# Autodesk Inventor assembly: Frame
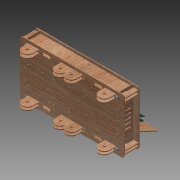
[picture p0: Inventor's stored thumbnail of the model, 180x180]
Saved by Autodesk Inventor 2015 (Build 190159000, 159)
## iProperties
Created: 2015-12-19
Part Number: Frame
Document SubType Name: Assembly
Designer: david
Author: david
## Documents named in this file (8)
- Z:\gip\Inventor\generatie 7\Frame\Frame.iam
- Z:\gip\Inventor\generatie 7\Frame\Electronica\Electronica.iam
- Z:\gip\Inventor\generatie 7\Frame\doos\zijiplaaten.ipt
- Z:\gip\Inventor\generatie 7\Frame\doos\voor-plaat.ipt
- Z:\gip\Inventor\generatie 7\Frame\afscherming.iam
- Z:\gip\Inventor\generatie 7\Frame\doos\TussenPalet.ipt
- Z:\gip\Inventor\generatie 7\Frame\vijs\vijs.ipt
- Z:\gip\Inventor\generatie 7\Frame\vijs\Moer.ipt
## Components (17 placed, 7 different names)
1. zijiplaaten:1 — Mate:26, Mate:35, Angle:1
2. zijiplaaten:2 — Mate:27
3. zijiplaaten:3 — Mate:20, Mate:36, Flush:3
4. zijiplaaten:4 — Mate:29, Mate:30, Mate:31, Flush:2
5. voor-plaat:1 — Flush:1, Mate:33
6. voor-plaat:2 — Mate:30, Mate:31, Mate:34
7. Electronica:1 [sub-assembly] — Mate:26, Mate:27, Mate:29, Mate:37, Mate:50, Mate:52, Mate:54, Mate:56
8. afscherming:1 [sub-assembly] — Mate:20, Mate:35, Mate:36, Flush:2, Flush:3, Mate:38, Mate:39, Mate:41, Mate:43, Mate:44, Mate:45, Mate:48
9. TussenPalet:1 — Flush:1, Mate:33, Mate:34
10. vijs:1 — Mate:37, Mate:38, Mate:49
11. vijs:2 — Mate:39, Mate:41, Mate:55
12. vijs:4 — Mate:43, Mate:44, Mate:51
13. vijs:5 — Mate:45, Mate:48, Mate:53
14. Moer:1 — Mate:49, Mate:50, Angle:1
15. Moer:2 — Mate:51, Mate:52
16. Moer:3 — Mate:53, Mate:54
17. Moer:4 — Mate:55, Mate:56
## Relationships (42: Mate 38, Flush 3, Angle 1)
- [Mate]: zijiplaaten:1 ↔ Electronica:1
- [Mate]: zijiplaaten:1 ↔ Electronica:1
- [Mate] (0.25 mm): zijiplaaten:2 ↔ Electronica:1
- [Mate] (2 mm): zijiplaaten:2 ↔ Electronica:1
- [Mate]: zijiplaaten:2 ↔ Electronica:1
- [Mate]: zijiplaaten:3 ↔ Electronica:1
- [Mate]: zijiplaaten:4 ↔ Electronica:1
- [Mate]: zijiplaaten:4 ↔ Electronica:1
- [Mate] (0.25 mm): zijiplaaten:1 ↔ voor-plaat:1
- [Mate] (0.25 mm): zijiplaaten:1 ↔ voor-plaat:1
- [Mate]: voor-plaat:1 ↔ Electronica:1
- [Mate]: voor-plaat:2 ↔ Electronica:1
- Mate:20: zijiplaaten:3 ↔ afscherming:1
- Mate:26 (2 mm): zijiplaaten:1 ↔ Electronica:1
- Mate:27 (2 mm): zijiplaaten:2 ↔ Electronica:1
- Mate:29 (2 mm): zijiplaaten:4 ↔ Electronica:1
- Mate:30 (0.25 mm): zijiplaaten:4 ↔ voor-plaat:2
- Mate:31 (0.25 mm): zijiplaaten:4 ↔ voor-plaat:2
- Flush:1: voor-plaat:1 ↔ TussenPalet:1
- Mate:33 (1 mm): voor-plaat:1 ↔ TussenPalet:1
- Mate:34: voor-plaat:2 ↔ TussenPalet:1
- Mate:35 (0.15 mm): zijiplaaten:1 ↔ afscherming:1
- Mate:36 (0.15 mm): zijiplaaten:3 ↔ afscherming:1
- Flush:2: zijiplaaten:4 ↔ afscherming:1
- Flush:3: zijiplaaten:3 ↔ afscherming:1
- Mate:37: Electronica:1 ↔ vijs:1
- Mate:38: afscherming:1 ↔ vijs:1
- Mate:39: afscherming:1 ↔ vijs:2
- Mate:41: afscherming:1 ↔ vijs:2
- Mate:43: afscherming:1 ↔ vijs:4
- Mate:44: afscherming:1 ↔ vijs:4
- Mate:45: afscherming:1 ↔ vijs:5
- Mate:48: afscherming:1 ↔ vijs:5
- Mate:49: vijs:1 ↔ Moer:1
- Mate:50: Electronica:1 ↔ Moer:1
- Angle:1 (0 deg): zijiplaaten:1 ↔ Moer:1
- Mate:51: vijs:4 ↔ Moer:2
- Mate:52: Electronica:1 ↔ Moer:2
- Mate:53: vijs:5 ↔ Moer:3
- Mate:54: Electronica:1 ↔ Moer:3
- Mate:55: vijs:2 ↔ Moer:4
- Mate:56: Electronica:1 ↔ Moer:4
## Named parameters: d8_d18 = 0 mm, d9_d19 = 0.25 mm, d10_d20 = 0.25 mm, d11_d21 = 0 mm, d13_d23 = 0 mm
